# Autodesk Inventor assembly: SwitchOnTNutHolderLeft
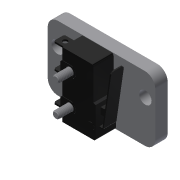
[picture p0: Inventor's stored thumbnail of the model, 180x180]
Saved by Autodesk Inventor 2018 (Build 220112000, 112)
## iProperties
Created: 2018-12-19
Part Number: SwitchOnTNutHolderLeft
Document SubType Name: Assembly
Designer: ball
Author: ball
## Documents named in this file (4)
- C:\FTC\FTC8863CAD\2018Robot\SwitchOnTNutHolderLeft.iam
- C:\FTC\FTC8863CAD\Actobotics\605 parts\605630.ipt
- C:\FTC\FTC8863CAD\2018Robot\SwitchHolderTNutLeft.ipt
- C:\FTC\FTC8863CAD\StepLibraries\Screws\2-56x.5_18-8 SS PAN HEAD PHILLIPS MACHINE SCREW.ipt
## Components (4 placed, 3 different names)
1. 605630:1 — Mate:1, Mate:2, Mate:3
2. SwitchHolderTNutLeft:1 — Mate:1, Mate:2, Mate:3, Mate:5, Mate:6, Mate:7, Mate:8
3. 2-56x.5_18-8 SS PAN HEAD PHILLIPS MACHINE SCREW:1 — Mate:7, Mate:8
4. 2-56x.5_18-8 SS PAN HEAD PHILLIPS MACHINE SCREW:2 — Mate:5, Mate:6
## Relationships (7: Mate 7)
- Mate:1: 605630:1 ↔ SwitchHolderTNutLeft:1
- Mate:2: 605630:1 ↔ SwitchHolderTNutLeft:1
- Mate:3: 605630:1 ↔ SwitchHolderTNutLeft:1
- Mate:5: SwitchHolderTNutLeft:1 ↔ 2-56x.5_18-8 SS PAN HEAD PHILLIPS MACHINE SCREW:2
- Mate:6: SwitchHolderTNutLeft:1 ↔ 2-56x.5_18-8 SS PAN HEAD PHILLIPS MACHINE SCREW:2
- Mate:7: SwitchHolderTNutLeft:1 ↔ 2-56x.5_18-8 SS PAN HEAD PHILLIPS MACHINE SCREW:1
- Mate:8: SwitchHolderTNutLeft:1 ↔ 2-56x.5_18-8 SS PAN HEAD PHILLIPS MACHINE SCREW:1
